# Autodesk Inventor assembly: Corner Z Axis Drag Chain
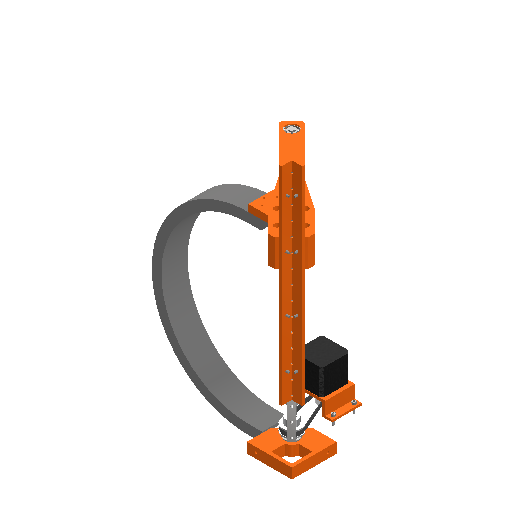
[picture p0: Inventor's stored thumbnail of the model, 512x512]
Saved by Autodesk Inventor 2023.2 (Build 272271000, 271)
## iProperties
Created: 2023-02-15
Part Number: Corner Z Axis Drag Chain
Document SubType Name: Assembly
Designer: remop
Author: remop
## Documents named in this file (20)
- C:\Users\remop\OneDrive\Documents\Inventor\3D Printers\LuEVO\Mk5_FullKinematic\Z Axis v2\Front left and right\Corner Z Axis Drag Chain.iam
- C:\Users\remop\OneDrive\Documents\Inventor\3D Printers\LuEVO\Mk5_FullKinematic\Z Axis v2\Front left and right\Corner Z Brace.ipt
- C:\Users\remop\OneDrive\Documents\Inventor\3D Printers\LuEVO\Mk5_FullKinematic\Z Axis v2\Drivetrain\MGN9H.ipt
- C:\Users\remop\OneDrive\Documents\Inventor\3D Printers\LuEVO\Mk5_FullKinematic\Z Axis v2\Drivetrain\MGNR9_300mm.ipt
- C:\Users\remop\OneDrive\Documents\Inventor\3D Printers\LuEVO\Mk5_FullKinematic\Z Axis v2\Front left and right\Corner Z Brace w Bearing.ipt
- C:\Users\remop\OneDrive\Documents\Inventor\3D Printers\LuEVO\Mk5_FullKinematic\Z Axis v2\Drivetrain\Z Axis Ball Screw.ipt
- C:\Users\remop\OneDrive\Documents\Inventor\Content Center Files\R2023\en-US\BS 290 SKF(21)\BS 290 SKF - SKF 608-RS1.ipt
- C:\Users\remop\OneDrive\Documents\Inventor\3D Printers\LuEVO\Mk5_FullKinematic\Z Axis v2\Drivetrain\Z Axis Ball Screw Bearing.ipt
- C:\Users\remop\OneDrive\Documents\Inventor\3D Printers\LuEVO\Mk5_FullKinematic\Z Axis v2\Front left and right\Z Axis Bottom Bearing Holder.ipt
- C:\Users\remop\OneDrive\Documents\Inventor\Content Center Files\R2023\en-US\AS 1420\AS 1420 - 1973 - M3 x 12.ipt
- C:\Users\remop\OneDrive\Documents\Inventor\Content Center Files\R2023\en-US\AS 1420\AS 1420 - 1973 - M3 x 8.ipt
- C:\Users\remop\OneDrive\Documents\Inventor\3D Printers\LuEVO\Mk5_FullKinematic\Z Axis v2\Drivetrain\Z Axis Belt Pulley.ipt
- C:\Users\remop\OneDrive\Documents\Inventor\3D Printers\LuEVO\Mk5_FullKinematic\Z Axis v2\WobbleX WS12.ipt
- C:\Users\remop\OneDrive\Documents\Inventor\3D Printers\LuEVO\Mk5_FullKinematic\Z Axis v2\WobbleX WS12 Bottom.ipt
- C:\Users\remop\OneDrive\Documents\Inventor\3D Printers\LuEVO\Mk5_FullKinematic\Z Axis v2\Front left and right\Corner Z Axis Carriage Drag Chain.ipt
- C:\Users\remop\OneDrive\Documents\Inventor\3D Printers\LuEVO\Mk5_FullKinematic\Z Axis v2\Front left and right\Z Drag Chain Dummy.ipt
- C:\Users\remop\OneDrive\Documents\Inventor\3D Printers\LuEVO\Mk5_FullKinematic\Z Axis v2\Drivetrain\Z Axis Belt.ipt
- C:\Users\remop\OneDrive\Documents\Inventor\3D Printers\LuEVO\Mk5_FullKinematic\Z Axis v2\Drivetrain\Z Axis Motor (Stepper).ipt
- C:\Users\remop\OneDrive\Documents\Inventor\3D Printers\LuEVO\Mk5_FullKinematic\XY Motion System\Belt Drives\Belt Pulley.ipt
- C:\Users\remop\OneDrive\Documents\Inventor\3D Printers\LuEVO\Mk5_FullKinematic\Z Axis v2\Drivetrain\Z Axis Motor Bracket.ipt
## Components (53 placed, 19 different names)
1. Corner Z Brace:1 — Flush:1, Mate:5, Mate:6, Rigid:1, Insert:18, Insert:19, Insert:22, Insert:23
2. MGN9H:1 — Mate:3, Mate:4, Angle:1, Flush:2, Rigid:6
3. MGNR9_300mm:1 — Mate:3, Mate:4, Flush:1, Mate:5, Mate:6, Insert:1, Insert:2, Insert:3, Insert:4, Insert:5, Insert:6, Insert:7, Insert:8, Insert:9, Insert:10, Insert:11, Insert:12, Insert:13, Insert:14, Insert:15
4. Corner Z Brace w Bearing:1 — Rigid:1, Rigid:2, Insert:16, Insert:17, Insert:20, Insert:21
5. Z Axis Ball Screw:1 — Rigid:3, Rigid:4, Mate:7, Rigid:5, Flush:5
6. BS 290 SKF- with RS1 seal SKF 608-RS1:1 — Rigid:2, Rigid:3
7. BS 290 SKF- with RS1 seal SKF 608-RS1:2 — Rigid:4, Rotational:1
8. Z Axis Ball Screw Bearing:1 — Mate:7, Angle:1, Flush:2, Rotational:2, Flush:3, Flush:5
9. Z Axis Bottom Bearing Holder:1 — Rotational:1, Flush:7
10. AS 1420 - Metric M3 x 12:1 — Insert:1
11. AS 1420 - Metric M3 x 12:2 — Insert:2
12. AS 1420 - Metric M3 x 12:3 — Insert:3
13. AS 1420 - Metric M3 x 12:4 — Insert:4
14. AS 1420 - Metric M3 x 12:5 — Insert:5
15. AS 1420 - Metric M3 x 12:6 — Insert:6
16. AS 1420 - Metric M3 x 12:7 — Insert:7
17. AS 1420 - Metric M3 x 12:8 — Insert:8
18. AS 1420 - Metric M3 x 12:9 — Insert:9
19. AS 1420 - Metric M3 x 12:10 — Insert:10
20. AS 1420 - Metric M3 x 12:11 — Insert:11
21. AS 1420 - Metric M3 x 12:12 — Insert:12
22. AS 1420 - Metric M3 x 12:13 — Insert:13
23. AS 1420 - Metric M3 x 12:14 — Insert:14
24. AS 1420 - Metric M3 x 12:15 — Insert:15
25. AS 1420 - Metric M3 x 8:1 — Insert:16
26. AS 1420 - Metric M3 x 8:2 — Insert:17
27. AS 1420 - Metric M3 x 8:3 — Insert:18
28. AS 1420 - Metric M3 x 8:4 — Insert:19
29. AS 1420 - Metric M3 x 8:5 — Insert:20
30. AS 1420 - Metric M3 x 8:6 — Insert:21
31. AS 1420 - Metric M3 x 8:7 — Insert:22
32. AS 1420 - Metric M3 x 8:8 — Insert:23
33. Z Axis Belt Pulley:1 — Rigid:5, Rotational:3
34. WobbleX WS12:1 — Rotational:2
35. WobbleX WS12 Bottom:1 — Flush:3
36. AS 1420 - Metric M3 x 8:9
37. AS 1420 - Metric M3 x 8:10
38. AS 1420 - Metric M3 x 8:11
39. AS 1420 - Metric M3 x 8:12
40. Corner Z Axis Carriage Drag Chain:1 — Rigid:6, Flush:6
41. Z Drag Chain Dummy:1 — Flush:6
42. Z Axis Belt:1 — Rotational:3, Rotational:4
43. Z Axis Motor (Stepper):2 — Flush:7, Rotational:4, Rotational:5, Rigid:7
44. Belt Pulley:1 — Rotational:5
45. Z Axis Motor Bracket:1 — Rigid:7, Insert:24, Insert:25, Insert:26, Insert:27, Insert:28, Insert:29, Insert:30, Insert:31
46. AS 1420 - Metric M3 x 8:13 — Insert:24
47. AS 1420 - Metric M3 x 8:14 — Insert:25
48. AS 1420 - Metric M3 x 8:15 — Insert:26
49. AS 1420 - Metric M3 x 8:16 — Insert:27
50. AS 1420 - Metric M3 x 12:16 — Insert:28
51. AS 1420 - Metric M3 x 12:17 — Insert:29
52. AS 1420 - Metric M3 x 12:18 — Insert:30
53. AS 1420 - Metric M3 x 12:19 — Insert:31
## Relationships (55: Insert 31, WeldJoint 7, Flush 6, Mate 5, RevoluteJoint 5, Angle 1)
- Mate:3: MGN9H:1 ↔ MGNR9_300mm:1
- Mate:4: MGN9H:1 ↔ MGNR9_300mm:1
- Flush:1 (-60 mm): Corner Z Brace:1 ↔ MGNR9_300mm:1
- Mate:5: Corner Z Brace:1 ↔ MGNR9_300mm:1
- Mate:6 (5.5 mm): Corner Z Brace:1 ↔ MGNR9_300mm:1
- Rigid:1 [WeldJoint]: Corner Z Brace:1 ↔ Corner Z Brace w Bearing:1
- Rigid:2 [WeldJoint]: Corner Z Brace w Bearing:1 ↔ BS 290 SKF- with RS1 seal SKF 608-RS1:1
- Rigid:3 [WeldJoint] (1 mm): Z Axis Ball Screw:1 ↔ BS 290 SKF- with RS1 seal SKF 608-RS1:1
- Rigid:4 [WeldJoint]: Z Axis Ball Screw:1 ↔ BS 290 SKF- with RS1 seal SKF 608-RS1:2
- Mate:7: Z Axis Ball Screw:1 ↔ Z Axis Ball Screw Bearing:1
- Angle:1 (0 deg): MGN9H:1 ↔ Z Axis Ball Screw Bearing:1
- Rotational:1 [RevoluteJoint]: BS 290 SKF- with RS1 seal SKF 608-RS1:2 ↔ Z Axis Bottom Bearing Holder:1
- Insert:1: MGNR9_300mm:1 ↔ AS 1420 - Metric M3 x 12:1
- Insert:2: MGNR9_300mm:1 ↔ AS 1420 - Metric M3 x 12:2
- Insert:3: MGNR9_300mm:1 ↔ AS 1420 - Metric M3 x 12:3
- Insert:4: MGNR9_300mm:1 ↔ AS 1420 - Metric M3 x 12:4
- Insert:5: MGNR9_300mm:1 ↔ AS 1420 - Metric M3 x 12:5
- Insert:6: MGNR9_300mm:1 ↔ AS 1420 - Metric M3 x 12:6
- Insert:7: MGNR9_300mm:1 ↔ AS 1420 - Metric M3 x 12:7
- Insert:8: MGNR9_300mm:1 ↔ AS 1420 - Metric M3 x 12:8
- Insert:9: MGNR9_300mm:1 ↔ AS 1420 - Metric M3 x 12:9
- Insert:10: MGNR9_300mm:1 ↔ AS 1420 - Metric M3 x 12:10
- Insert:11: MGNR9_300mm:1 ↔ AS 1420 - Metric M3 x 12:11
- Insert:12: MGNR9_300mm:1 ↔ AS 1420 - Metric M3 x 12:12
- Insert:13: MGNR9_300mm:1 ↔ AS 1420 - Metric M3 x 12:13
- Insert:14: MGNR9_300mm:1 ↔ AS 1420 - Metric M3 x 12:14
- Insert:15: MGNR9_300mm:1 ↔ AS 1420 - Metric M3 x 12:15
- Insert:16: Corner Z Brace w Bearing:1 ↔ AS 1420 - Metric M3 x 8:1
- Insert:17: Corner Z Brace w Bearing:1 ↔ AS 1420 - Metric M3 x 8:2
- Insert:18: Corner Z Brace:1 ↔ AS 1420 - Metric M3 x 8:3
- Insert:19: Corner Z Brace:1 ↔ AS 1420 - Metric M3 x 8:4
- Insert:20: Corner Z Brace w Bearing:1 ↔ AS 1420 - Metric M3 x 8:5
- Insert:21: Corner Z Brace w Bearing:1 ↔ AS 1420 - Metric M3 x 8:6
- Insert:22: Corner Z Brace:1 ↔ AS 1420 - Metric M3 x 8:7
- Insert:23: Corner Z Brace:1 ↔ AS 1420 - Metric M3 x 8:8
- Rigid:5 [WeldJoint] (-5 mm): Z Axis Ball Screw:1 ↔ Z Axis Belt Pulley:1
- Flush:2: MGN9H:1 ↔ Z Axis Ball Screw Bearing:1
- Rotational:2 [RevoluteJoint] (-8 mm): Z Axis Ball Screw Bearing:1 ↔ WobbleX WS12:1
- Flush:3: Z Axis Ball Screw Bearing:1 ↔ WobbleX WS12 Bottom:1
- Flush:5 (200 mm): Z Axis Ball Screw:1 ↔ Z Axis Ball Screw Bearing:1
- Rigid:6 [WeldJoint]: MGN9H:1 ↔ Corner Z Axis Carriage Drag Chain:1
- Flush:6: Corner Z Axis Carriage Drag Chain:1 ↔ Z Drag Chain Dummy:1
- Rotational:3 [RevoluteJoint]: Z Axis Belt Pulley:1 ↔ Z Axis Belt:1
- Flush:7 (40 mm): Z Axis Bottom Bearing Holder:1 ↔ Z Axis Motor (Stepper):2
- Rotational:4 [RevoluteJoint] (-9.35 mm): Z Axis Belt:1 ↔ Z Axis Motor (Stepper):2
- Rotational:5 [RevoluteJoint] (0.5 mm): Z Axis Motor (Stepper):2 ↔ Belt Pulley:1
- Rigid:7 [WeldJoint]: Z Axis Motor (Stepper):2 ↔ Z Axis Motor Bracket:1
- Insert:24: Z Axis Motor Bracket:1 ↔ AS 1420 - Metric M3 x 8:13
- Insert:25: Z Axis Motor Bracket:1 ↔ AS 1420 - Metric M3 x 8:14
- Insert:26: Z Axis Motor Bracket:1 ↔ AS 1420 - Metric M3 x 8:15
- Insert:27: Z Axis Motor Bracket:1 ↔ AS 1420 - Metric M3 x 8:16
- Insert:28: Z Axis Motor Bracket:1 ↔ AS 1420 - Metric M3 x 12:16
- Insert:29: Z Axis Motor Bracket:1 ↔ AS 1420 - Metric M3 x 12:17
- Insert:30: Z Axis Motor Bracket:1 ↔ AS 1420 - Metric M3 x 12:18
- Insert:31: Z Axis Motor Bracket:1 ↔ AS 1420 - Metric M3 x 12:19
